# Autodesk Inventor assembly: ASSEMBLY_X_axis_carriage
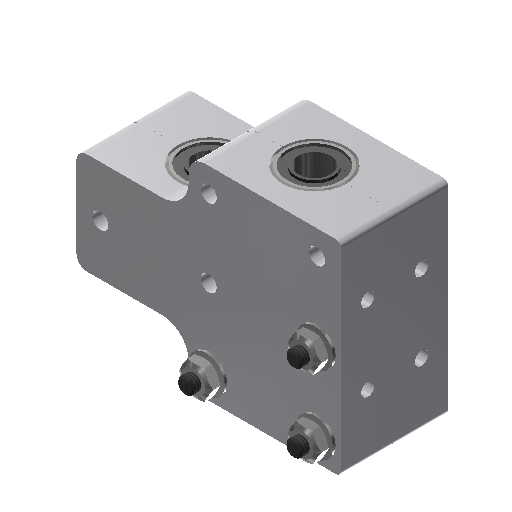
[picture p0: Inventor's stored thumbnail of the model, 512x512]
Saved by Autodesk Inventor 2026.1 (Build 301233000, 233)
## iProperties
Created: 2018-07-08
Part Number: ASSEMBLY_X_axis_carriage
Document SubType Name: Assembly
Designer: Andrzej
Author: Andrzej
## Documents named in this file (6)
- C:\Users\Andrzej\OneDrive\_DRIVE_SYNCH_FILES\__ BYTECHLAB PROJECTS\MLTDIS - SMD Parts Sorting Machine\MCAD\1_REV1\ASSEMBLY_XY_AXIS_REVA\ASSEMBLY_X_axis_carriage.iam
- C:\Users\Andrzej\OneDrive\_DRIVE_SYNCH_FILES\__ BYTECHLAB PROJECTS\MLTDIS - SMD Parts Sorting Machine\MCAD\1_REV1\__COTS_PARTS\COTS_GENERIC_LMM6UU_Linear_bearing.ipt
- C:\Users\Andrzej\OneDrive\_DRIVE_SYNCH_FILES\__ BYTECHLAB PROJECTS\MLTDIS - SMD Parts Sorting Machine\MCAD\1_REV1\ASSEMBLY_XY_AXIS_REVA\3DP_PLA_X_axis_carriage_half.ipt
- C:\Users\Andrzej\OneDrive\_DRIVE_SYNCH_FILES\__ BYTECHLAB PROJECTS\MLTDIS - SMD Parts Sorting Machine\MCAD\1_REV1\__CONTENT_CENTER_PARTS\en-US\DIN 125-2  A\DIN 125-2 - A 3,2A.ipt
- C:\Users\Andrzej\OneDrive\_DRIVE_SYNCH_FILES\__ BYTECHLAB PROJECTS\MLTDIS - SMD Parts Sorting Machine\MCAD\1_REV1\__CONTENT_CENTER_PARTS\en-US\ISO 7380-1\ISO 7380-1 - M3 x 25.ipt
- C:\Users\Andrzej\OneDrive\_DRIVE_SYNCH_FILES\__ BYTECHLAB PROJECTS\MLTDIS - SMD Parts Sorting Machine\MCAD\1_REV1\__CONTENT_CENTER_PARTS\en-US\DIN 934\DIN 934 - M3 x 0,5.ipt
## Components (17 placed, 5 different names)
1. COTS_GENERIC_LMM6UU_Linear_bearing:1 — Mate:3, Mate:4
2. COTS_GENERIC_LMM6UU_Linear_bearing:2 — Mate:5, Flush:4
3. COTS_GENERIC_LMM6UU_Linear_bearing:3 — Mate:2, Mate:4, Flush:3
4. 3DP_PLA_X_axis_carriage_half:1 — Mate:1, Flush:1, Flush:2, Mate:2, Mate:3, Flush:3, Mate:5, Mate:10, Mate:11, Mate:12, Mate:13, Mate:14, Mate:15, Mate:20, Mate:22, Mate:24
5. 3DP_PLA_X_axis_carriage_half:2 — Mate:1, Flush:1, Flush:2, Flush:4, Mate:21, Mate:23, Mate:25
6. DIN 125-2 A A 3,2:4 — Mate:10, Mate:11, Insert:3
7. DIN 125-2 A A 3,2:5 — Mate:12, Mate:13, Insert:4
8. DIN 125-2 A A 3,2:6 — Mate:14, Mate:15, Insert:5
9. ISO 7380-1 M3 x 25:3 — Insert:3
10. ISO 7380-1 M3 x 25:4 — Insert:4
11. ISO 7380-1 M3 x 25:5 — Insert:5
12. DIN 125-2 A A 3,2:8 — Mate:20, Mate:21, Insert:8
13. DIN 125-2 A A 3,2:9 — Mate:22, Mate:23, Insert:9
14. DIN 125-2 A A 3,2:10 — Mate:24, Mate:25, Insert:10
15. DIN 934 - replaced by DIN EN 24032/28673/28674 M3:3 — Insert:8
16. DIN 934 - replaced by DIN EN 24032/28673/28674 M3:4 — Insert:9
17. DIN 934 - replaced by DIN EN 24032/28673/28674 M3:5 — Insert:10
## Relationships (27: Mate 17, Insert 6, Flush 4)
- Mate:1: 3DP_PLA_X_axis_carriage_half:1 ↔ 3DP_PLA_X_axis_carriage_half:2
- Flush:1: 3DP_PLA_X_axis_carriage_half:1 ↔ 3DP_PLA_X_axis_carriage_half:2
- Flush:2: 3DP_PLA_X_axis_carriage_half:1 ↔ 3DP_PLA_X_axis_carriage_half:2
- Mate:2: COTS_GENERIC_LMM6UU_Linear_bearing:3 ↔ 3DP_PLA_X_axis_carriage_half:1
- Mate:3: COTS_GENERIC_LMM6UU_Linear_bearing:1 ↔ 3DP_PLA_X_axis_carriage_half:1
- Mate:4: COTS_GENERIC_LMM6UU_Linear_bearing:1 ↔ COTS_GENERIC_LMM6UU_Linear_bearing:3
- Flush:3: COTS_GENERIC_LMM6UU_Linear_bearing:3 ↔ 3DP_PLA_X_axis_carriage_half:1
- Mate:5: COTS_GENERIC_LMM6UU_Linear_bearing:2 ↔ 3DP_PLA_X_axis_carriage_half:1
- Flush:4: COTS_GENERIC_LMM6UU_Linear_bearing:2 ↔ 3DP_PLA_X_axis_carriage_half:2
- Mate:10: 3DP_PLA_X_axis_carriage_half:1 ↔ DIN 125-2 A A 3,2:4
- Mate:11: 3DP_PLA_X_axis_carriage_half:1 ↔ DIN 125-2 A A 3,2:4
- Mate:12: 3DP_PLA_X_axis_carriage_half:1 ↔ DIN 125-2 A A 3,2:5
- Mate:13: 3DP_PLA_X_axis_carriage_half:1 ↔ DIN 125-2 A A 3,2:5
- Mate:14: 3DP_PLA_X_axis_carriage_half:1 ↔ DIN 125-2 A A 3,2:6
- Mate:15: 3DP_PLA_X_axis_carriage_half:1 ↔ DIN 125-2 A A 3,2:6
- Insert:3: DIN 125-2 A A 3,2:4 ↔ ISO 7380-1 M3 x 25:3
- Insert:4: DIN 125-2 A A 3,2:5 ↔ ISO 7380-1 M3 x 25:4
- Insert:5: DIN 125-2 A A 3,2:6 ↔ ISO 7380-1 M3 x 25:5
- Mate:20: 3DP_PLA_X_axis_carriage_half:1 ↔ DIN 125-2 A A 3,2:8
- Mate:21: 3DP_PLA_X_axis_carriage_half:2 ↔ DIN 125-2 A A 3,2:8
- Mate:22: 3DP_PLA_X_axis_carriage_half:1 ↔ DIN 125-2 A A 3,2:9
- Mate:23: 3DP_PLA_X_axis_carriage_half:2 ↔ DIN 125-2 A A 3,2:9
- Mate:24: 3DP_PLA_X_axis_carriage_half:1 ↔ DIN 125-2 A A 3,2:10
- Mate:25: 3DP_PLA_X_axis_carriage_half:2 ↔ DIN 125-2 A A 3,2:10
- Insert:8: DIN 125-2 A A 3,2:8 ↔ DIN 934 - replaced by DIN EN 24032/28673/28674 M3:3
- Insert:9: DIN 125-2 A A 3,2:9 ↔ DIN 934 - replaced by DIN EN 24032/28673/28674 M3:4
- Insert:10: DIN 125-2 A A 3,2:10 ↔ DIN 934 - replaced by DIN EN 24032/28673/28674 M3:5
